# Autodesk Inventor assembly: EnsambleMecanismoEnsayo
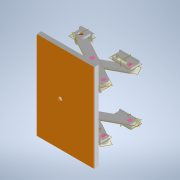
[picture p0: Inventor's stored thumbnail of the model, 180x180]
Saved by Autodesk Inventor 2021 (Build 250183000, 183)
## iProperties
Created: 2021-04-17
Part Number: EnsambleMecanismoEnsayo
Document SubType Name: Assembly
Designer: GABRIEL LOL
Author: GABRIEL LOL
## Documents named in this file (9)
- C:\Users\GABRIEL LOL\OneDrive - Universidad Nacional de Colombia\PAI\3_Producto 3D\EnsambleMecanismoEnsayo.iam
- C:\Users\GABRIEL LOL\OneDrive - Universidad Nacional de Colombia\PAI\3_Producto 3D\PasadorPivotePreliminar.ipt
- C:\Users\GABRIEL LOL\OneDrive - Universidad Nacional de Colombia\PAI\3_Producto 3D\PasadorPreliminar.ipt
- C:\Users\GABRIEL LOL\OneDrive - Universidad Nacional de Colombia\PAI\3_Producto 3D\EslabonPreliminarElevacion.ipt
- C:\Users\GABRIEL LOL\OneDrive - Universidad Nacional de Colombia\PAI\3_Producto 3D\ApoyoRotatorioPreliminar.ipt
- C:\Users\GABRIEL LOL\OneDrive - Universidad Nacional de Colombia\PAI\3_Producto 3D\PistaEslabonPreliminar.ipt
- C:\Users\GABRIEL LOL\OneDrive - Universidad Nacional de Colombia\PAI\3_Producto 3D\SoporteBaseElevacion.ipt
- C:\Users\GABRIEL LOL\OneDrive - Universidad Nacional de Colombia\PAI\3_Producto 3D\BaseExtrusion.ipt
- C:\Users\GABRIEL LOL\OneDrive - Universidad Nacional de Colombia\PAI\3_Producto 3D\PisoDeEnsayoIgnorar.ipt
## Components (25 placed, 8 different names)
1. PasadorPivotePreliminar:1 — Mate:31, Flush:16, Mate:32
2. EslabonPreliminarElevacion:1 — Mate:18, Flush:9, Mate:26, Flush:11, Mate:29, Flush:15, Flush:24
3. ApoyoRotatorioPreliminar:1 — Mate:32, Flush:17, Mate:33, Flush:21
4. EslabonPreliminarElevacion:2 — Mate:3, Mate:4, Mate:6, Mate:13, Flush:6, Mate:28, Flush:19
5. EslabonPreliminarElevacion:3 — Mate:12, Flush:5, Mate:25, Flush:10, Mate:31, Flush:16, Flush:17
6. EslabonPreliminarElevacion:4 — Mate:14, Mate:15, Flush:7, Mate:17, Flush:8, Mate:27, Flush:18
7. ApoyoRotatorioPreliminar:2 — Mate:30, Flush:14, Flush:15, Mate:34, Flush:20
8. ApoyoRotatorioPreliminar:3 — Mate:2, Mate:7, Flush:3, Mate:14, Mate:16
9. ApoyoRotatorioPreliminar:4 — Mate:1, Mate:5, Mate:6, Mate:7, Flush:2, Flush:3, Flush:4, Mate:21, Mate:22
10. PasadorPivotePreliminar:2 — Mate:29, Mate:30, Flush:14
11. PasadorPivotePreliminar:3 — Mate:15, Flush:7, Mate:16
12. PasadorPivotePreliminar:4 — Mate:3, Mate:4, Mate:5
13. PasadorPreliminar:2 — Mate:17, Flush:8, Mate:18, Flush:9
14. PasadorPreliminar:3 — Mate:12, Mate:13, Flush:5, Flush:6
15. PistaEslabonPreliminar:1 — Mate:20, Mate:23, Mate:24, Transitional:3, Transitional:4
16. PistaEslabonPreliminar:2 — Mate:19, Mate:21, Mate:22, Mate:23, Mate:24, Transitional:1, Transitional:2, Flush:25
17. SoporteBaseElevacion:1 — Mate:8, Mate:9, Mate:10, Mate:33, Mate:34, Mate:35, Mate:36, Flush:20, Flush:21
18. BaseExtrusion:1 — Mate:8, Mate:9, Mate:10
19. PisoDeEnsayoIgnorar:1 — Mate:1, Mate:2, Flush:2, Flush:4, Mate:19, Mate:20
20. PistaEslabonPreliminar:3 — Transitional:5, Transitional:6, Mate:35, Flush:22, Flush:23, Flush:25
21. PistaEslabonPreliminar:4 — Mate:36, Flush:22, Flush:23, Flush:24
22. PasadorPreliminar:4 — Mate:25, Flush:10, Transitional:1, Transitional:2
23. PasadorPreliminar:6 — Mate:26, Flush:11, Transitional:3, Transitional:4
24. PasadorPreliminar:7 — Mate:28, Flush:19, Transitional:5, Transitional:6
25. PasadorPreliminar:8 — Mate:27, Flush:18
## Relationships (63: Mate 35, Flush 22, Transitional 6)
- Mate:1: ApoyoRotatorioPreliminar:4 ↔ PisoDeEnsayoIgnorar:1
- Mate:2: ApoyoRotatorioPreliminar:3 ↔ PisoDeEnsayoIgnorar:1
- Mate:3: EslabonPreliminarElevacion:2 ↔ PasadorPivotePreliminar:4
- Mate:4: EslabonPreliminarElevacion:2 ↔ PasadorPivotePreliminar:4
- Mate:5: ApoyoRotatorioPreliminar:4 ↔ PasadorPivotePreliminar:4
- Mate:6: EslabonPreliminarElevacion:2 ↔ ApoyoRotatorioPreliminar:4
- Mate:7: ApoyoRotatorioPreliminar:3 ↔ ApoyoRotatorioPreliminar:4
- Mate:8: SoporteBaseElevacion:1 ↔ BaseExtrusion:1
- Mate:9: SoporteBaseElevacion:1 ↔ BaseExtrusion:1
- Mate:10: SoporteBaseElevacion:1 ↔ BaseExtrusion:1
- Flush:2: ApoyoRotatorioPreliminar:4 ↔ PisoDeEnsayoIgnorar:1
- Flush:3 (250 mm): ApoyoRotatorioPreliminar:3 ↔ ApoyoRotatorioPreliminar:4
- Flush:4 (108 mm): ApoyoRotatorioPreliminar:4 ↔ PisoDeEnsayoIgnorar:1
- Mate:12: EslabonPreliminarElevacion:3 ↔ PasadorPreliminar:3
- Mate:13: EslabonPreliminarElevacion:2 ↔ PasadorPreliminar:3
- Flush:5: EslabonPreliminarElevacion:3 ↔ PasadorPreliminar:3
- Flush:6: EslabonPreliminarElevacion:2 ↔ PasadorPreliminar:3
- Mate:14: EslabonPreliminarElevacion:4 ↔ ApoyoRotatorioPreliminar:3
- Mate:15: EslabonPreliminarElevacion:4 ↔ PasadorPivotePreliminar:3
- Flush:7: EslabonPreliminarElevacion:4 ↔ PasadorPivotePreliminar:3
- Mate:16: ApoyoRotatorioPreliminar:3 ↔ PasadorPivotePreliminar:3
- Mate:17: EslabonPreliminarElevacion:4 ↔ PasadorPreliminar:2
- Flush:8: EslabonPreliminarElevacion:4 ↔ PasadorPreliminar:2
- Mate:18: EslabonPreliminarElevacion:1 ↔ PasadorPreliminar:2
- Flush:9: EslabonPreliminarElevacion:1 ↔ PasadorPreliminar:2
- Mate:19: PistaEslabonPreliminar:2 ↔ PisoDeEnsayoIgnorar:1
- Mate:20: PistaEslabonPreliminar:1 ↔ PisoDeEnsayoIgnorar:1
- Mate:21: ApoyoRotatorioPreliminar:4 ↔ PistaEslabonPreliminar:2
- Mate:22 (173.4 mm): ApoyoRotatorioPreliminar:4 ↔ PistaEslabonPreliminar:2
- Mate:23: PistaEslabonPreliminar:1 ↔ PistaEslabonPreliminar:2
- Mate:24 (-250 mm): PistaEslabonPreliminar:1 ↔ PistaEslabonPreliminar:2
- Mate:25: EslabonPreliminarElevacion:3 ↔ PasadorPreliminar:4
- Flush:10: EslabonPreliminarElevacion:3 ↔ PasadorPreliminar:4
- Transitional:1: PistaEslabonPreliminar:2 ↔ PasadorPreliminar:4
- Transitional:2: PistaEslabonPreliminar:2 ↔ PasadorPreliminar:4
- Mate:26: EslabonPreliminarElevacion:1 ↔ PasadorPreliminar:6
- Flush:11: EslabonPreliminarElevacion:1 ↔ PasadorPreliminar:6
- Transitional:3: PistaEslabonPreliminar:1 ↔ PasadorPreliminar:6
- Transitional:4: PistaEslabonPreliminar:1 ↔ PasadorPreliminar:6
- Mate:27: EslabonPreliminarElevacion:4 ↔ PasadorPreliminar:8
- Mate:28: EslabonPreliminarElevacion:2 ↔ PasadorPreliminar:7
- Mate:29: EslabonPreliminarElevacion:1 ↔ PasadorPivotePreliminar:2
- Mate:30: ApoyoRotatorioPreliminar:2 ↔ PasadorPivotePreliminar:2
- Flush:14: ApoyoRotatorioPreliminar:2 ↔ PasadorPivotePreliminar:2
- Flush:15: EslabonPreliminarElevacion:1 ↔ ApoyoRotatorioPreliminar:2
- Mate:31: PasadorPivotePreliminar:1 ↔ EslabonPreliminarElevacion:3
- Flush:16: PasadorPivotePreliminar:1 ↔ EslabonPreliminarElevacion:3
- Mate:32: PasadorPivotePreliminar:1 ↔ ApoyoRotatorioPreliminar:1
- Flush:17: ApoyoRotatorioPreliminar:1 ↔ EslabonPreliminarElevacion:3
- Flush:18: EslabonPreliminarElevacion:4 ↔ PasadorPreliminar:8
- Flush:19: EslabonPreliminarElevacion:2 ↔ PasadorPreliminar:7
- Transitional:5: PistaEslabonPreliminar:3 ↔ PasadorPreliminar:7
- Transitional:6: PistaEslabonPreliminar:3 ↔ PasadorPreliminar:7
- Mate:33: ApoyoRotatorioPreliminar:1 ↔ SoporteBaseElevacion:1
- Mate:34: ApoyoRotatorioPreliminar:2 ↔ SoporteBaseElevacion:1
- Mate:35: SoporteBaseElevacion:1 ↔ PistaEslabonPreliminar:3
- Mate:36: SoporteBaseElevacion:1 ↔ PistaEslabonPreliminar:4
- Flush:20: ApoyoRotatorioPreliminar:2 ↔ SoporteBaseElevacion:1
- Flush:21 (-105 mm): ApoyoRotatorioPreliminar:1 ↔ SoporteBaseElevacion:1
- Flush:22: PistaEslabonPreliminar:3 ↔ PistaEslabonPreliminar:4
- Flush:23 (220 mm): PistaEslabonPreliminar:3 ↔ PistaEslabonPreliminar:4
- Flush:24: EslabonPreliminarElevacion:1 ↔ PistaEslabonPreliminar:4
- Flush:25: PistaEslabonPreliminar:2 ↔ PistaEslabonPreliminar:3
